# Autodesk Inventor assembly: EnsamblajeCasa
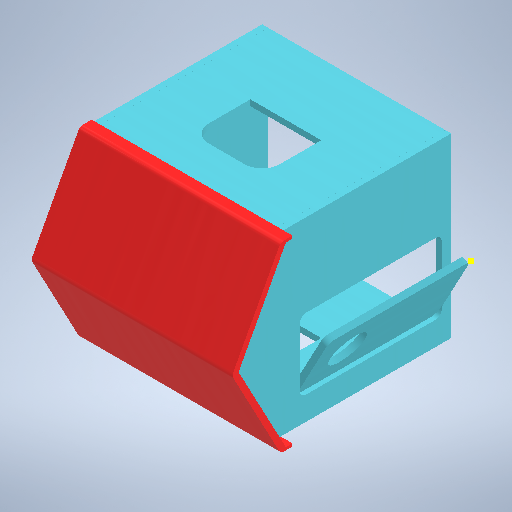
[picture p0: Inventor's stored thumbnail of the model, 512x512]
Saved by Autodesk Inventor 2025.1 (Build 291241000, 241)
## iProperties
Created: 2025-01-19
Part Number: EnsamblajeCasa
Document SubType Name: Assembly
Designer: usuario
Author: usuario
## Documents named in this file (6)
- C:\Users\yovan\Desktop\APM\ausol-apm.github.io\project\Design and simulation\Inventor\Modelado juguetes\Casa\EnsamblajeCasaFinal.iam
- C:\Users\yovan\Desktop\APM\ausol-apm.github.io\project\Design and simulation\Inventor\Modelado juguetes\Casa\ParedDelanteraCasa.ipt
- C:\Users\yovan\Desktop\APM\ausol-apm.github.io\project\Design and simulation\Inventor\Modelado juguetes\Casa\ParedLateralCasa.ipt
- C:\Users\yovan\Desktop\APM\ausol-apm.github.io\project\Design and simulation\Inventor\Modelado juguetes\Casa\ParedTraseraCasa.ipt
- C:\Users\yovan\Desktop\APM\ausol-apm.github.io\project\Design and simulation\Inventor\Modelado juguetes\Casa\Puerta.ipt
- C:\Users\yovan\Desktop\APM\ausol-apm.github.io\project\Design and simulation\Inventor\Modelado juguetes\Casa\TechoCasa.ipt
## Components (6 placed, 5 different names)
1. ParedDelanteraCasa:1 — Mate:1, Mate:2, Mate:5, Mate:6, Mate:7, Mate:8, Mate:9, Mate:10, Mate:12
2. ParedLateralCasa:1 — Mate:5, Mate:6
3. ParedTraseraCasa:1 — Mate:3, Mate:4, Flush:1, Mate:11, Flush:2
4. Puerta:1 — Mate:8, Mate:9
5. ParedLateralCasa:2 — Mate:1, Mate:2, Mate:3, Mate:4, Flush:1, Mate:7
6. TechoCasa:1 — Mate:10, Mate:11, Mate:12, Flush:2
## Relationships (14: Mate 12, Flush 2)
- Mate:1: ParedDelanteraCasa:1 ↔ ParedLateralCasa:2
- Mate:2: ParedDelanteraCasa:1 ↔ ParedLateralCasa:2
- Mate:3: ParedTraseraCasa:1 ↔ ParedLateralCasa:2
- Mate:4: ParedTraseraCasa:1 ↔ ParedLateralCasa:2
- Mate:5: ParedDelanteraCasa:1 ↔ ParedLateralCasa:1
- Mate:6: ParedDelanteraCasa:1 ↔ ParedLateralCasa:1
- Flush:1: ParedTraseraCasa:1 ↔ ParedLateralCasa:2
- Mate:7: ParedDelanteraCasa:1 ↔ ParedLateralCasa:2
- Mate:8: ParedDelanteraCasa:1 ↔ Puerta:1
- Mate:9: ParedDelanteraCasa:1 ↔ Puerta:1
- Mate:10: ParedDelanteraCasa:1 ↔ TechoCasa:1
- Mate:11: ParedTraseraCasa:1 ↔ TechoCasa:1
- Mate:12: ParedDelanteraCasa:1 ↔ TechoCasa:1
- Flush:2: ParedTraseraCasa:1 ↔ TechoCasa:1
